# Autodesk Inventor assembly: DT Side Assembly_MIR1
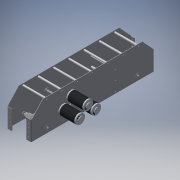
[picture p0: Inventor's stored thumbnail of the model, 180x180]
Saved by Autodesk Inventor 2016 (Build 200138000, 138)
## iProperties
Created: 2018-05-03
Part Number: DT Side Assembly_MIR1
Document SubType Name: Assembly
Designer: Kade
Mass: 2864.4 g
Surface Area: 10801.9 cm^2
Volume: 2767.29 cm^3
Density: 1.03509 g/cm^3
Author: 2000083068
## Documents named in this file (13)
- F:\Robotics\Off Season\Blannon\DT Side Assembly_MIR1.iam
- F:\Robotics\Off Season\Blannon\Fixed Side frame_MIR1.ipt
- F:\Robotics\Off Season\Blannon\72t_Aluminum_Spur_Gear_20_DP_1_2_Hex_Bore_217-3576_MIR1.ipt
- F:\Robotics\Off Season\Blannon\24t_Steel_Spur_Gear_20_DP_1_2_Hex_Bore_217-5464_MIR1.ipt
- F:\Robotics\Off Season\Blannon\Cim Motor_MIR1.ipt
- F:\Robotics\Off Season\Blannon\11t_Steel_Spur_Gear_20_DP_CIM_Motor_12t_Center_Distance_217-3107_MIR1.ipt
- F:\Robotics\Off Season\Blannon\.5 ID Flanged Bearing_MIR1.ipt
- F:\Robotics\Off Season\Blannon\ThunderHex_Stock_18in_MIR1.ipt
- F:\Robotics\Off Season\Blannon\Wheel Hub_MIR1.ipt
- F:\Robotics\Off Season\Blannon\30t_x_9mm_Wide_Double_Flange_Aluminum_Pulley_HTD_5mm_1_2_Hex_Bore_217-3229_MIR.ipt
- F:\Robotics\Off Season\Blannon\30t_x_15mm_Wide_Aluminum_Pulley_HTD_5mm_1_2_Hex_217-4102_MIR.ipt
- F:\Robotics\Off Season\Blannon\Fixed Side Frame Outside_MIR1.ipt
- F:\Robotics\Off Season\Blannon\Delrin Spacer_MIR.ipt
## Components (44 placed, 12 different names)
1. Fixed Side frame_MIR1:1 — Mate:89, Mate:88, Insert:17, Insert:18, Insert:19, Mate:81, Mate:80, Mate:77, Mate:76, Insert:15, Insert:16, Mate:79, Mate:78, Flush:30, Flush:29, Insert:34, Insert:33, Insert:32, Insert:31, Insert:30, Insert:29, Insert:28, Insert:27, Insert:26, Insert:25
2. 72t_Aluminum_Spur_Gear_20_DP_1_2_Hex_Bore_217-3576_MIR1:1 — Mate:71, Insert:14
3. 72t_Aluminum_Spur_Gear_20_DP_1_2_Hex_Bore_217-3576_MIR1:2 — Flush:19, Mate:75, Mate:74, Mate:94
4. 24t_Steel_Spur_Gear_20_DP_1_2_Hex_Bore_217-5464_MIR1:1 — Flush:19, Mate:71, Mate:73, Mate:72
5. Cim Motor_MIR1:1 — Insert:17, Flush:8, Mate:31
6. Cim Motor_MIR1:2 — Insert:18, Mate:67, Flush:18
7. Cim Motor_MIR1:3 — Insert:19, Flush:7, Mate:30
8. 11t_Steel_Spur_Gear_20_DP_CIM_Motor_12t_Center_Distance_217-3107_MIR1:1 — Mate:67, Flush:18
9. 11t_Steel_Spur_Gear_20_DP_CIM_Motor_12t_Center_Distance_217-3107_MIR1:2 — Flush:8, Mate:31
10. 11t_Steel_Spur_Gear_20_DP_CIM_Motor_12t_Center_Distance_217-3107_MIR1:3 — Flush:7, Mate:30
11. .5 ID Flanged Bearing_MIR1:1 — Mate:81, Mate:80, Insert:9
12. .5 ID Flanged Bearing_MIR1:2 — Mate:77, Mate:76, Insert:12
13. .5 ID Flanged Bearing_MIR1:3 — Insert:15, Insert:10
14. .5 ID Flanged Bearing_MIR1:4 — Insert:16, Insert:11
15. .5 ID Flanged Bearing_MIR1:5 — Mate:79, Mate:78, Insert:13
16. ThunderHex_Stock_18in_MIR1:1 — Mate:75, Mate:74, Insert:10, Mate:91, Mate:90
17. ThunderHex_Stock_18in_MIR1:2 — Mate:73, Mate:72, Insert:14, Insert:11
18. ThunderHex_Stock_18in_MIR1:3 — Insert:13, Mate:87, Mate:86, Mate:101, Mate:100
19. ThunderHex_Stock_18in_MIR1:4 — Insert:9, Mate:83, Mate:82, Mate:99, Mate:98
20. ThunderHex_Stock_18in_MIR1:5 — Insert:12, Mate:85, Mate:84, Mate:93, Mate:92, Mate:96, Mate:95
21. Wheel Hub_MIR1:1 — Mate:83, Mate:82, Flush:26, Flush:27, Mate:102
22. Wheel Hub_MIR1:2 — Flush:26, Mate:85, Mate:84
23. Wheel Hub_MIR1:3 — Flush:27, Mate:87, Mate:86
24. 30t_x_9mm_Wide_Double_Flange_Aluminum_Pulley_HTD_5mm_1_2_Hex_Bore_217-3229_MIR:1 — Mate:102, Mate:99, Mate:98, Flush:21
25. 30t_x_9mm_Wide_Double_Flange_Aluminum_Pulley_HTD_5mm_1_2_Hex_Bore_217-3229_MIR:2 — Mate:101, Mate:100, Flush:22
26. 30t_x_9mm_Wide_Double_Flange_Aluminum_Pulley_HTD_5mm_1_2_Hex_Bore_217-3229_MIR:3 — Mate:94, Mate:91, Mate:90, Flush:20
27. 30t_x_9mm_Wide_Double_Flange_Aluminum_Pulley_HTD_5mm_1_2_Hex_Bore_217-3229_MIR:4 — Flush:20, Mate:93, Mate:92, Mate:97
28. 30t_x_15mm_Wide_Aluminum_Pulley_HTD_5mm_1_2_Hex_217-4102_MIR:1 — Flush:22, Flush:21, Mate:97, Mate:96, Mate:95
29. Fixed Side Frame Outside_MIR1:1 — Flush:30, Flush:29
30. .5 ID Flanged Bearing_MIR1:6
31. .5 ID Flanged Bearing_MIR1:7
32. .5 ID Flanged Bearing_MIR1:8
33. .5 ID Flanged Bearing_MIR1:9
34. .5 ID Flanged Bearing_MIR1:10
35. Delrin Spacer_MIR:1 — Insert:34
36. Delrin Spacer_MIR:2 — Insert:33
37. Delrin Spacer_MIR:3 — Insert:32
38. Delrin Spacer_MIR:4 — Insert:31
39. Delrin Spacer_MIR:5 — Insert:30
40. Delrin Spacer_MIR:6 — Insert:29
41. Delrin Spacer_MIR:7 — Insert:28
42. Delrin Spacer_MIR:8 — Insert:27
43. Delrin Spacer_MIR:9 — Insert:26
44. Delrin Spacer_MIR:10 — Insert:25
## Relationships (67: Mate 34, Insert 21, Flush 12)
- Mate:89: Fixed Side frame_MIR1:1
- Mate:88 [Flush]: Fixed Side frame_MIR1:1
- Flush:19: 72t_Aluminum_Spur_Gear_20_DP_1_2_Hex_Bore_217-3576_MIR1:2 ↔ 24t_Steel_Spur_Gear_20_DP_1_2_Hex_Bore_217-5464_MIR1:1
- Mate:71: 72t_Aluminum_Spur_Gear_20_DP_1_2_Hex_Bore_217-3576_MIR1:1 ↔ 24t_Steel_Spur_Gear_20_DP_1_2_Hex_Bore_217-5464_MIR1:1
- Insert:17 (3.175 mm): Fixed Side frame_MIR1:1 ↔ Cim Motor_MIR1:1
- Insert:18 (3.175 mm): Fixed Side frame_MIR1:1 ↔ Cim Motor_MIR1:2
- Insert:19 (3.175 mm): Fixed Side frame_MIR1:1 ↔ Cim Motor_MIR1:3
- Mate:67: Cim Motor_MIR1:2 ↔ 11t_Steel_Spur_Gear_20_DP_CIM_Motor_12t_Center_Distance_217-3107_MIR1:1
- Flush:18 (3.175 mm): Cim Motor_MIR1:2 ↔ 11t_Steel_Spur_Gear_20_DP_CIM_Motor_12t_Center_Distance_217-3107_MIR1:1
- Flush:8 (-3.175 mm): Cim Motor_MIR1:1 ↔ 11t_Steel_Spur_Gear_20_DP_CIM_Motor_12t_Center_Distance_217-3107_MIR1:2
- Mate:31: Cim Motor_MIR1:1 ↔ 11t_Steel_Spur_Gear_20_DP_CIM_Motor_12t_Center_Distance_217-3107_MIR1:2
- Flush:7 (-3.175 mm): Cim Motor_MIR1:3 ↔ 11t_Steel_Spur_Gear_20_DP_CIM_Motor_12t_Center_Distance_217-3107_MIR1:3
- Mate:30: Cim Motor_MIR1:3 ↔ 11t_Steel_Spur_Gear_20_DP_CIM_Motor_12t_Center_Distance_217-3107_MIR1:3
- Mate:81: Fixed Side frame_MIR1:1 ↔ .5 ID Flanged Bearing_MIR1:1
- Mate:80: Fixed Side frame_MIR1:1 ↔ .5 ID Flanged Bearing_MIR1:1
- Mate:77: Fixed Side frame_MIR1:1 ↔ .5 ID Flanged Bearing_MIR1:2
- Mate:76: Fixed Side frame_MIR1:1 ↔ .5 ID Flanged Bearing_MIR1:2
- Insert:15 (-6.35 mm): Fixed Side frame_MIR1:1 ↔ .5 ID Flanged Bearing_MIR1:3
- Insert:16: Fixed Side frame_MIR1:1 ↔ .5 ID Flanged Bearing_MIR1:4
- Mate:79: Fixed Side frame_MIR1:1 ↔ .5 ID Flanged Bearing_MIR1:5
- Mate:78: Fixed Side frame_MIR1:1 ↔ .5 ID Flanged Bearing_MIR1:5
- Mate:75: 72t_Aluminum_Spur_Gear_20_DP_1_2_Hex_Bore_217-3576_MIR1:2 ↔ ThunderHex_Stock_18in_MIR1:1
- Mate:74: 72t_Aluminum_Spur_Gear_20_DP_1_2_Hex_Bore_217-3576_MIR1:2 ↔ ThunderHex_Stock_18in_MIR1:1
- Insert:10: .5 ID Flanged Bearing_MIR1:3 ↔ ThunderHex_Stock_18in_MIR1:1
- Mate:73: 24t_Steel_Spur_Gear_20_DP_1_2_Hex_Bore_217-5464_MIR1:1 ↔ ThunderHex_Stock_18in_MIR1:2
- Mate:72: 24t_Steel_Spur_Gear_20_DP_1_2_Hex_Bore_217-5464_MIR1:1 ↔ ThunderHex_Stock_18in_MIR1:2
- Insert:14 (-25.4 mm): 72t_Aluminum_Spur_Gear_20_DP_1_2_Hex_Bore_217-3576_MIR1:1 ↔ ThunderHex_Stock_18in_MIR1:2
- Insert:11: .5 ID Flanged Bearing_MIR1:4 ↔ ThunderHex_Stock_18in_MIR1:2
- Insert:13: .5 ID Flanged Bearing_MIR1:5 ↔ ThunderHex_Stock_18in_MIR1:3
- Insert:9: .5 ID Flanged Bearing_MIR1:1 ↔ ThunderHex_Stock_18in_MIR1:4
- Insert:12 (6.35 mm): .5 ID Flanged Bearing_MIR1:2 ↔ ThunderHex_Stock_18in_MIR1:5
- Mate:83: ThunderHex_Stock_18in_MIR1:4 ↔ Wheel Hub_MIR1:1
- Mate:82: ThunderHex_Stock_18in_MIR1:4 ↔ Wheel Hub_MIR1:1
- Flush:26: Wheel Hub_MIR1:1 ↔ Wheel Hub_MIR1:2
- Mate:85: ThunderHex_Stock_18in_MIR1:5 ↔ Wheel Hub_MIR1:2
- Mate:84: ThunderHex_Stock_18in_MIR1:5 ↔ Wheel Hub_MIR1:2
- Flush:27: Wheel Hub_MIR1:1 ↔ Wheel Hub_MIR1:3
- Mate:87: ThunderHex_Stock_18in_MIR1:3 ↔ Wheel Hub_MIR1:3
- Mate:86: ThunderHex_Stock_18in_MIR1:3 ↔ Wheel Hub_MIR1:3
- Mate:102 (3.175 mm): Wheel Hub_MIR1:1 ↔ 30t_x_9mm_Wide_Double_Flange_Aluminum_Pulley_HTD_5mm_1_2_Hex_Bore_217-3229_MIR:1
- Mate:99: ThunderHex_Stock_18in_MIR1:4 ↔ 30t_x_9mm_Wide_Double_Flange_Aluminum_Pulley_HTD_5mm_1_2_Hex_Bore_217-3229_MIR:1
- Mate:98: ThunderHex_Stock_18in_MIR1:4 ↔ 30t_x_9mm_Wide_Double_Flange_Aluminum_Pulley_HTD_5mm_1_2_Hex_Bore_217-3229_MIR:1
- Mate:101: ThunderHex_Stock_18in_MIR1:3 ↔ 30t_x_9mm_Wide_Double_Flange_Aluminum_Pulley_HTD_5mm_1_2_Hex_Bore_217-3229_MIR:2
- Mate:100: ThunderHex_Stock_18in_MIR1:3 ↔ 30t_x_9mm_Wide_Double_Flange_Aluminum_Pulley_HTD_5mm_1_2_Hex_Bore_217-3229_MIR:2
- Mate:94 (3.175 mm): 72t_Aluminum_Spur_Gear_20_DP_1_2_Hex_Bore_217-3576_MIR1:2 ↔ 30t_x_9mm_Wide_Double_Flange_Aluminum_Pulley_HTD_5mm_1_2_Hex_Bore_217-3229_MIR:3
- Mate:91: ThunderHex_Stock_18in_MIR1:1 ↔ 30t_x_9mm_Wide_Double_Flange_Aluminum_Pulley_HTD_5mm_1_2_Hex_Bore_217-3229_MIR:3
- Mate:90: ThunderHex_Stock_18in_MIR1:1 ↔ 30t_x_9mm_Wide_Double_Flange_Aluminum_Pulley_HTD_5mm_1_2_Hex_Bore_217-3229_MIR:3
- Flush:20: 30t_x_9mm_Wide_Double_Flange_Aluminum_Pulley_HTD_5mm_1_2_Hex_Bore_217-3229_MIR:3 ↔ 30t_x_9mm_Wide_Double_Flange_Aluminum_Pulley_HTD_5mm_1_2_Hex_Bore_217-3229_MIR:4
- Mate:93: ThunderHex_Stock_18in_MIR1:5 ↔ 30t_x_9mm_Wide_Double_Flange_Aluminum_Pulley_HTD_5mm_1_2_Hex_Bore_217-3229_MIR:4
- Mate:92: ThunderHex_Stock_18in_MIR1:5 ↔ 30t_x_9mm_Wide_Double_Flange_Aluminum_Pulley_HTD_5mm_1_2_Hex_Bore_217-3229_MIR:4
- Flush:22: 30t_x_9mm_Wide_Double_Flange_Aluminum_Pulley_HTD_5mm_1_2_Hex_Bore_217-3229_MIR:2 ↔ 30t_x_15mm_Wide_Aluminum_Pulley_HTD_5mm_1_2_Hex_217-4102_MIR:1
- Flush:21: 30t_x_9mm_Wide_Double_Flange_Aluminum_Pulley_HTD_5mm_1_2_Hex_Bore_217-3229_MIR:1 ↔ 30t_x_15mm_Wide_Aluminum_Pulley_HTD_5mm_1_2_Hex_217-4102_MIR:1
- Mate:97: 30t_x_9mm_Wide_Double_Flange_Aluminum_Pulley_HTD_5mm_1_2_Hex_Bore_217-3229_MIR:4 ↔ 30t_x_15mm_Wide_Aluminum_Pulley_HTD_5mm_1_2_Hex_217-4102_MIR:1
- Mate:96: ThunderHex_Stock_18in_MIR1:5 ↔ 30t_x_15mm_Wide_Aluminum_Pulley_HTD_5mm_1_2_Hex_217-4102_MIR:1
- Mate:95: ThunderHex_Stock_18in_MIR1:5 ↔ 30t_x_15mm_Wide_Aluminum_Pulley_HTD_5mm_1_2_Hex_217-4102_MIR:1
- Flush:30: Fixed Side frame_MIR1:1 ↔ Fixed Side Frame Outside_MIR1:1
- Flush:29: Fixed Side frame_MIR1:1 ↔ Fixed Side Frame Outside_MIR1:1
- Insert:34: Fixed Side frame_MIR1:1 ↔ Delrin Spacer_MIR:1
- Insert:33: Fixed Side frame_MIR1:1 ↔ Delrin Spacer_MIR:2
- Insert:32: Fixed Side frame_MIR1:1 ↔ Delrin Spacer_MIR:3
- Insert:31: Fixed Side frame_MIR1:1 ↔ Delrin Spacer_MIR:4
- Insert:30: Fixed Side frame_MIR1:1 ↔ Delrin Spacer_MIR:5
- Insert:29: Fixed Side frame_MIR1:1 ↔ Delrin Spacer_MIR:6
- Insert:28: Fixed Side frame_MIR1:1 ↔ Delrin Spacer_MIR:7
- Insert:27: Fixed Side frame_MIR1:1 ↔ Delrin Spacer_MIR:8
- Insert:26: Fixed Side frame_MIR1:1 ↔ Delrin Spacer_MIR:9
- Insert:25: Fixed Side frame_MIR1:1 ↔ Delrin Spacer_MIR:10
